# Autodesk Inventor assembly: two_servo_frame_with_nuts
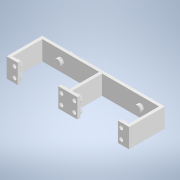
[picture p0: Inventor's stored thumbnail of the model, 180x180]
Saved by Autodesk Inventor 2021.4 (Build 254397000, 397)
## iProperties
Created: 2022-07-24
Part Number: two_servo_frame_with_nuts
Document SubType Name: Assembly
Designer: isamu
Author: isamu
## Documents named in this file (4)
- D:\personal_projects\robot\inventor\2021_matlab_compat _v2\servo_frames\two_servo_frame_with_nuts.iam
- D:\personal_projects\robot\exports\screws\m4 nuts.ipt
- D:\personal_projects\robot\exports\frames\two_servo_frame_combined.ipt
- D:\personal_projects\robot\exports\screws\m4x12.ipt
## Components (13 placed, 3 different names)
1. m4 nuts:1 — Insert:4
2. m4 nuts:2 — Insert:2
3. m4 nuts:3 — Insert:1
4. m4 nuts:4 — Insert:3
5. two_servo_frame_combined:1 — Insert:1, Insert:2, Insert:3, Insert:4, Insert:5, Insert:6, Insert:7, Insert:8, Insert:9, Insert:10, Insert:11, Insert:12
6. m4 nuts:5 — Insert:5
7. m4 nuts:6 — Insert:6
8. m4 nuts:7 — Insert:7
9. m4 nuts:8 — Insert:8
10. m4 nuts:9 — Insert:10
11. m4 nuts:10 — Insert:9
12. m4x12:1 — Insert:11
13. m4x12:2 — Insert:12
## Relationships (12: Insert 12)
- Insert:1: m4 nuts:3 ↔ two_servo_frame_combined:1
- Insert:2: m4 nuts:2 ↔ two_servo_frame_combined:1
- Insert:3: m4 nuts:4 ↔ two_servo_frame_combined:1
- Insert:4: m4 nuts:1 ↔ two_servo_frame_combined:1
- Insert:5: two_servo_frame_combined:1 ↔ m4 nuts:5
- Insert:6: two_servo_frame_combined:1 ↔ m4 nuts:6
- Insert:7: two_servo_frame_combined:1 ↔ m4 nuts:7
- Insert:8: two_servo_frame_combined:1 ↔ m4 nuts:8
- Insert:9: two_servo_frame_combined:1 ↔ m4 nuts:10
- Insert:10: two_servo_frame_combined:1 ↔ m4 nuts:9
- Insert:11: two_servo_frame_combined:1 ↔ m4x12:1
- Insert:12: two_servo_frame_combined:1 ↔ m4x12:2
